# Autodesk Inventor assembly: Ensamble_Termoformadora
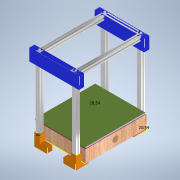
[picture p0: Inventor's stored thumbnail of the model, 180x180]
Saved by Autodesk Inventor 2022.6 (Build 266554000, 554)
## iProperties
Created: 2025-02-18
Part Number: Ensamble_Termoformadora
Document SubType Name: Assembly
Designer: johan
Author: johan
## Documents named in this file (9)
- D:\RutasNew\Desktop\Termoformadora\Ensamble_Termoformadora.iam
- D:\RutasNew\Desktop\Termoformadora\MADERA.ipt
- D:\RutasNew\Desktop\Termoformadora\Fomi.ipt
- D:\RutasNew\Desktop\Termoformadora\rejilla.ipt
- D:\RutasNew\Desktop\Termoformadora\Perfil400mm.ipt
- D:\RutasNew\Desktop\Termoformadora\esquina20mm.ipt
- D:\RutasNew\Desktop\Termoformadora\Perfil300mm.ipt
- D:\RutasNew\Desktop\Termoformadora\Perfil146mm.ipt
- D:\RutasNew\Desktop\Termoformadora\Travesaño.ipt
## Components (21 placed, 8 different names)
1. MADERA:1 — Coincidencia:2, Nivelación:1, Nivelación:2, Coincidencia:4, Coincidencia:5, Coincidencia:7, Coincidencia:8, Coincidencia:10, Coincidencia:11, Coincidencia:13, Coincidencia:14
2. Fomi:1 — Coincidencia:2, Nivelación:1, Nivelación:2, Coincidencia:3, Nivelación:3, Nivelación:4
3. rejilla:1 — Coincidencia:3, Nivelación:3, Nivelación:4
4. esquina20mm:1 — Coincidencia:4, Coincidencia:5, Coincidencia:6
5. Perfil400mm:1 — Coincidencia:6, Coincidencia:17, Coincidencia:23
6. esquina20mm:2 — Coincidencia:7, Coincidencia:8, Coincidencia:9
7. Perfil400mm:2 — Coincidencia:9, Coincidencia:18
8. esquina20mm:3 — Coincidencia:10, Coincidencia:11, Coincidencia:12
9. esquina20mm:4 — Coincidencia:13, Coincidencia:14, Coincidencia:15
10. Perfil400mm:3 — Coincidencia:12, Coincidencia:16, Coincidencia:20, Coincidencia:21, Coincidencia:24, Coincidencia:25
11. Perfil400mm:4 — Coincidencia:15, Coincidencia:19, Coincidencia:22, Coincidencia:26, Coincidencia:27
12. esquina20mm:5 — Coincidencia:16
13. esquina20mm:6 — Coincidencia:19
14. esquina20mm:7 — Coincidencia:18
15. esquina20mm:8 — Coincidencia:17
16. Perfil300mm:1 — Coincidencia:20
17. Perfil300mm:2 — Coincidencia:23
18. Perfil146mm:1 — Coincidencia:21
19. Perfil146mm:2 — Coincidencia:22
20. Travesaño:1 — Coincidencia:24, Coincidencia:25
21. Travesaño:2 — Coincidencia:26, Coincidencia:27
## Relationships (30: Mate 26, Flush 4)
- Coincidencia:2 [Mate]: MADERA:1 ↔ Fomi:1
- Nivelación:1 [Flush]: MADERA:1 ↔ Fomi:1
- Nivelación:2 [Flush]: MADERA:1 ↔ Fomi:1
- Coincidencia:3 [Mate]: Fomi:1 ↔ rejilla:1
- Nivelación:3 [Flush]: Fomi:1 ↔ rejilla:1
- Nivelación:4 [Flush]: Fomi:1 ↔ rejilla:1
- Coincidencia:4 [Mate]: MADERA:1 ↔ esquina20mm:1
- Coincidencia:5 [Mate]: MADERA:1 ↔ esquina20mm:1
- Coincidencia:6 [Mate]: esquina20mm:1 ↔ Perfil400mm:1
- Coincidencia:7 [Mate]: MADERA:1 ↔ esquina20mm:2
- Coincidencia:8 [Mate]: MADERA:1 ↔ esquina20mm:2
- Coincidencia:9 [Mate]: esquina20mm:2 ↔ Perfil400mm:2
- Coincidencia:10 [Mate]: MADERA:1 ↔ esquina20mm:3
- Coincidencia:11 [Mate]: MADERA:1 ↔ esquina20mm:3
- Coincidencia:12 [Mate]: esquina20mm:3 ↔ Perfil400mm:3
- Coincidencia:13 [Mate]: MADERA:1 ↔ esquina20mm:4
- Coincidencia:14 [Mate]: MADERA:1 ↔ esquina20mm:4
- Coincidencia:15 [Mate]: esquina20mm:4 ↔ Perfil400mm:4
- Coincidencia:16 [Mate]: Perfil400mm:3 ↔ esquina20mm:5
- Coincidencia:17 [Mate]: Perfil400mm:1 ↔ esquina20mm:8
- Coincidencia:18 [Mate]: Perfil400mm:2 ↔ esquina20mm:7
- Coincidencia:19 [Mate]: Perfil400mm:4 ↔ esquina20mm:6
- Coincidencia:20 [Mate]: Perfil400mm:3 ↔ Perfil300mm:1
- Coincidencia:21 [Mate]: Perfil400mm:3 ↔ Perfil146mm:1
- Coincidencia:22 [Mate]: Perfil400mm:4 ↔ Perfil146mm:2
- Coincidencia:23 [Mate]: Perfil400mm:1 ↔ Perfil300mm:2
- Coincidencia:24 [Mate]: Perfil400mm:3 ↔ Travesaño:1
- Coincidencia:25 [Mate]: Perfil400mm:3 ↔ Travesaño:1
- Coincidencia:26 [Mate]: Perfil400mm:4 ↔ Travesaño:2
- Coincidencia:27 [Mate]: Perfil400mm:4 ↔ Travesaño:2
